# Autodesk Inventor assembly: Pump-Motor-CW-Rotation:Diaphragrm Pump
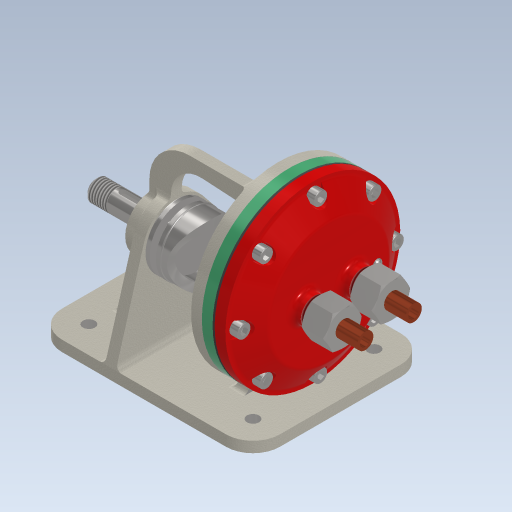
[picture p0: Inventor's stored thumbnail of the model, 512x512]
Saved by Autodesk Inventor 2024.2 (Build 282272000, 272)
## iProperties
Created: 2025-06-16
Document SubType Name: Assembly
Designer: cw
Description: Diaphragrm Pump
Author: cw
## Documents named in this file (18)
- C:\zWSA2025 TP05 M1\Solution\Diaphragrm Pump Final.iam
- C:\zWSA2025 TP05 M1\Solution\Pump\Base.ipt
- C:\zWSA2025 TP05 M1\Solution\Pump\Case 102.ipt
- C:\zWSA2025 TP05 M1\Solution\Pump\Diaphragm.ipt
- C:\zWSA2025 TP05 M1\Solution\Pump\Case 101.ipt
- C:\zWSA2025 TP05 M1\Solution\Pump\Valve 101.ipt
- C:\zWSA2025 TP05 M1\Solution\Pump\ISO_R 1051 - 4 x 18 x 9.5.ipt
- C:\zWSA2025 TP05 M1\Solution\Pump\Valve 102.ipt
- C:\zWSA2025 TP05 M1\Solution\Pump\Pipe.ipt
- C:\zWSA2025 TP05 M1\Solution\Pump\Spring 102.ipt
- C:\zWSA2025 TP05 M1\Solution\Pump\Union Nut.ipt
- C:\zWSA2025 TP05 M1\Solution\Content Center\en-US\ISO 4762(2)\ISO 4762 - M6 x 25ISO.ipt
- C:\zWSA2025 TP05 M1\Solution\Pump\Follower.ipt
- C:\zWSA2025 TP05 M1\Solution\Content Center\en-US\ISO 104\ISO 104 - 3 73 - 20 x 47 x 12.ipt
- C:\zWSA2025 TP05 M1\Solution\Content Center\en-US\DIN 625 SKF(5)\DIN 625 SKF - SKF 61804-2RS1.ipt
- C:\zWSA2025 TP05 M1\Solution\Pump\Spring 101.ipt
- C:\zWSA2025 TP05 M1\Solution\Cam Shaft\Cam Shaft-2x010.ipt
- C:\zWSA2025 TP05 M1\Solution\Cam Shaft.ipt
## Components (25 placed, 16 different names)
1. Base:1 — Mate:1, Mate:2, Mate:3, Mate:28, Angle:2(RotateCam)
2. Case 102:1 — Mate:1, Mate:2, Mate:3, Mate:4, Mate:5, Mate:6, Mate:15, Mate:16, Mate:22, Flush:11
3. Diaphragm:1 — Mate:4, Mate:5, Mate:6, Mate:17
4. Case 101:1 — Mate:7, Mate:8, Flush:1, Mate:9, Mate:10, Mate:11, Mate:12, Mate:13, Flush:2, Mate:14, Flush:3, Mate:15, Mate:16, Mate:17, Flush:4, Flush:5, Mate:18, Mate:19, Mate:20, Mate:21, Angle:1
5. Valve 101:1 — Mate:7, Mate:8, Flush:1
6. ISO_R 1051 - 4 x 18 x 9.5:1 — Mate:9, Mate:10
7. Valve 102:1 — Mate:11, Mate:12, Flush:6, Flush:7, Flush:8
8. Pipe:1 — Mate:13, Flush:2, Flush:4, Flush:10
9. Pipe:2 — Mate:14, Flush:3, Flush:5, Flush:6, Flush:9
10. Spring 102:1 — Flush:7, Flush:8, Flush:9
11. Follower:1 — Mate:22, Flush:11, Tangent:1, Flush:12
12. DIN 625 SKF- with two RS1 seals SKF 61804-2RS1:1 — Mate:31, Mate:33
13. ISO 104 (Single Direction) 3 73 - 20 x 47 x 12:1 — Mate:28, Mate:29, Mate:30, Angle:3
14. Cam Shaft-2x010:1 — Mate:29, Mate:30, Mate:31, Tangent:1, Angle:2(RotateCam), Mate:33, Angle:3
15. Spring 101:1 — Flush:12
16. Union Nut:1 — Mate:18, Mate:19, Flush:10
17. Union Nut:2
18. ISO 4762 M6 x 25:1 — Mate:20, Mate:21, Angle:1
19. ISO 4762 M6 x 25:2
20. ISO 4762 M6 x 25:3
21. ISO 4762 M6 x 25:4
22. ISO 4762 M6 x 25:5
23. ISO 4762 M6 x 25:6
24. ISO 4762 M6 x 25:7
25. ISO 4762 M6 x 25:8
## Component patterns: (2 elements, first: Union Nut:1), (8 elements, first: ISO 4762 M6 x 25:1)
## Relationships (45: Mate 29, Flush 12, Angle 3, Tangent 1)
- Mate:1: Base:1 ↔ Case 102:1
- Mate:2: Base:1 ↔ Case 102:1
- Mate:3: Base:1 ↔ Case 102:1
- Mate:4: Case 102:1 ↔ Diaphragm:1
- Mate:5: Case 102:1 ↔ Diaphragm:1
- Mate:6: Case 102:1 ↔ Diaphragm:1
- Mate:7: Case 101:1 ↔ Valve 101:1
- Mate:8: Case 101:1 ↔ Valve 101:1
- Flush:1: Case 101:1 ↔ Valve 101:1
- Mate:9: Case 101:1 ↔ ISO_R 1051 - 4 x 18 x 9.5:1
- Mate:10: Case 101:1 ↔ ISO_R 1051 - 4 x 18 x 9.5:1
- Mate:11: Case 101:1 ↔ Valve 102:1
- Mate:12: Case 101:1 ↔ Valve 102:1
- Mate:13: Case 101:1 ↔ Pipe:1
- Flush:2: Case 101:1 ↔ Pipe:1
- Mate:14: Case 101:1 ↔ Pipe:2
- Flush:3: Case 101:1 ↔ Pipe:2
- Mate:15: Case 102:1 ↔ Case 101:1
- Mate:16: Case 102:1 ↔ Case 101:1
- Mate:17: Diaphragm:1 ↔ Case 101:1
- Flush:4: Case 101:1 ↔ Pipe:1
- Flush:5: Case 101:1 ↔ Pipe:2
- Flush:6: Valve 102:1 ↔ Pipe:2
- Flush:7: Valve 102:1 ↔ Spring 102:1
- Flush:8: Valve 102:1 ↔ Spring 102:1
- Flush:9: Pipe:2 ↔ Spring 102:1
- Mate:18: Case 101:1 ↔ Union Nut:1
- Mate:19: Case 101:1 ↔ Union Nut:1
- Flush:10: Pipe:1 ↔ Union Nut:1
- Mate:20: Case 101:1 ↔ ISO 4762 M6 x 25:1
- Mate:21: Case 101:1 ↔ ISO 4762 M6 x 25:1
- Angle:1 (0 deg): Case 101:1 ↔ ISO 4762 M6 x 25:1
- Mate:22: Case 102:1 ↔ Follower:1
- Flush:11: Case 102:1 ↔ Follower:1
- [Mate]: Base:1 ↔ DIN 625 SKF- with two RS1 seals SKF 61804-2RS1:1
- [Mate]: Base:1 ↔ DIN 625 SKF- with two RS1 seals SKF 61804-2RS1:1
- Mate:28: Base:1 ↔ ISO 104 (Single Direction) 3 73 - 20 x 47 x 12:1
- Mate:29: ISO 104 (Single Direction) 3 73 - 20 x 47 x 12:1 ↔ Cam Shaft-2x010:1
- Mate:30: ISO 104 (Single Direction) 3 73 - 20 x 47 x 12:1 ↔ Cam Shaft-2x010:1
- Mate:31: DIN 625 SKF- with two RS1 seals SKF 61804-2RS1:1 ↔ Cam Shaft-2x010:1
- Tangent:1: Follower:1 ↔ Cam Shaft-2x010:1
- Angle:2(RotateCam) (0 deg): Base:1 ↔ Cam Shaft-2x010:1
- Flush:12: Follower:1 ↔ Spring 101:1
- Mate:33: DIN 625 SKF- with two RS1 seals SKF 61804-2RS1:1 ↔ Cam Shaft-2x010:1
- Angle:3 (0 deg): ISO 104 (Single Direction) 3 73 - 20 x 47 x 12:1 ↔ Cam Shaft-2x010:1
